# Autodesk Inventor assembly: Assembly
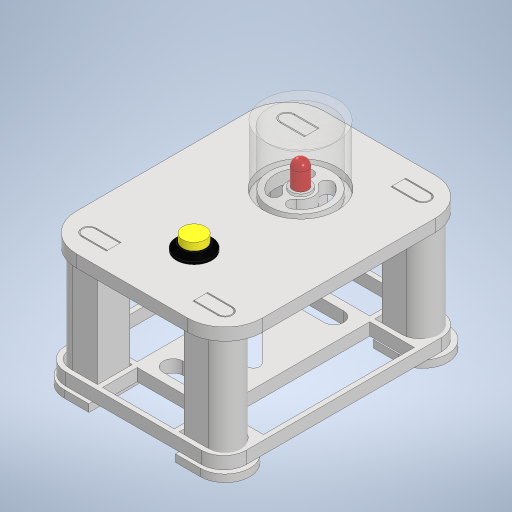
[picture p0: Inventor's stored thumbnail of the model, 512x512]
Saved by Autodesk Inventor 2024.1 (Build 281209000, 209)
## iProperties
Created: 2023-12-30
Part Number: Assembly
Document SubType Name: Assembly
Designer: ryanm
Author: ryanm
## Documents named in this file (8)
- C:\Users\ryanm\OneDrive - Colyton Grammar School\A-Levels\Other\Buzzer System\3D CAD\Slim Version\Assembly.iam
- C:\Users\ryanm\OneDrive - Colyton Grammar School\A-Levels\Other\Buzzer System\3D CAD\Slim Version\Plate.ipt
- C:\Users\ryanm\OneDrive - Colyton Grammar School\A-Levels\Other\Buzzer System\3D CAD\Slim Version\Stand.ipt
- C:\Users\ryanm\OneDrive - Colyton Grammar School\A-Levels\Other\Buzzer System\3D CAD\Slim Version\LED Cover.ipt
- C:\Users\ryanm\OneDrive - Colyton Grammar School\A-Levels\Other\Buzzer System\3D CAD\8mm Through-Hole LED.ipt
- C:\Users\ryanm\OneDrive - Colyton Grammar School\A-Levels\Other\Buzzer System\3D CAD\Microbit Breakout.ipt
- C:\Users\ryanm\OneDrive - Colyton Grammar School\A-Levels\Other\Buzzer System\3D CAD\Button.ipt
- C:\Users\ryanm\OneDrive - Colyton Grammar School\A-Levels\Other\Buzzer System\3D CAD\Slim Version\Stand Brace.ipt
## Components (10 placed, 7 different names)
1. Plate:1 — Mate:1, Mate:2, Mate:3, Flush:1, Mate:4, Flush:2, Mate:5, Flush:3, Flush:4, Mate:6, Mate:7, Mate:8, Mate:10, Mate:11, Flush:5, Flush:6, Mate:12, Mate:13
2. Stand:1 — Mate:3, Flush:1, Flush:7, Mate:14, Mate:15, Mate:16
3. Stand:2 — Mate:4, Flush:2, Flush:7
4. Stand:3 — Mate:5, Flush:3, Flush:8
5. Stand:4 — Flush:4, Mate:6, Flush:8
6. LED Cover:1 — Mate:9, Mate:10
7. 8mm Through-Hole LED:1 — Mate:7, Mate:8, Mate:9
8. Microbit Breakout:1 — Mate:11, Flush:5, Flush:6
9. Button:1 — Mate:12, Mate:13
10. Stand Brace:1 — Mate:14, Mate:15, Mate:16
## Relationships (24: Mate 16, Flush 8)
- Mate:1: Plate:1
- Mate:2: Plate:1
- Mate:3: Plate:1 ↔ Stand:1
- Flush:1: Plate:1 ↔ Stand:1
- Mate:4: Plate:1 ↔ Stand:2
- Flush:2: Plate:1 ↔ Stand:2
- Mate:5: Plate:1 ↔ Stand:3
- Flush:3: Plate:1 ↔ Stand:3
- Flush:4: Plate:1 ↔ Stand:4
- Mate:6: Plate:1 ↔ Stand:4
- Mate:7: Plate:1 ↔ 8mm Through-Hole LED:1
- Mate:8: Plate:1 ↔ 8mm Through-Hole LED:1
- Mate:9: LED Cover:1 ↔ 8mm Through-Hole LED:1
- Mate:10: Plate:1 ↔ LED Cover:1
- Mate:11: Plate:1 ↔ Microbit Breakout:1
- Flush:5 (10 mm): Plate:1 ↔ Microbit Breakout:1
- Flush:6 (22.5 mm): Plate:1 ↔ Microbit Breakout:1
- Mate:12: Plate:1 ↔ Button:1
- Mate:13: Plate:1 ↔ Button:1
- Flush:7: Stand:1 ↔ Stand:2
- Flush:8: Stand:3 ↔ Stand:4
- Mate:14: Stand:1 ↔ Stand Brace:1
- Mate:15: Stand:1 ↔ Stand Brace:1
- Mate:16: Stand:1 ↔ Stand Brace:1
